# Autodesk Inventor assembly: FrameV2
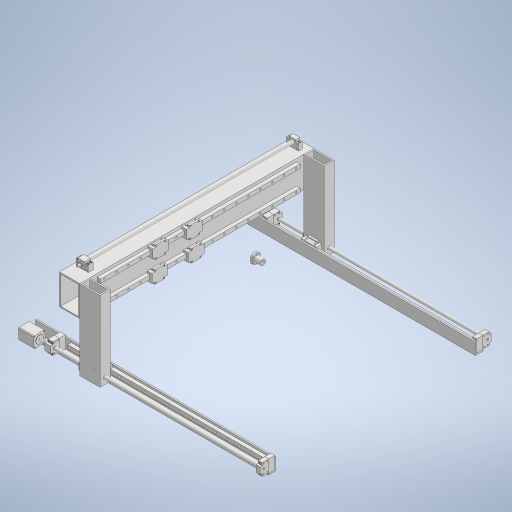
[picture p0: Inventor's stored thumbnail of the model, 512x512]
Saved by Autodesk Inventor 2023 (Build 270158000, 158)
## iProperties
Created: 2022-05-01
Part Number: FrameV2
Document SubType Name: Assembly
Designer: plebbb
Author: plebbb
## Documents named in this file (14)
- D:\Users\plebbb\Desktop\CNC_Project\FrameV2.iam
- D:\Users\plebbb\Desktop\CNC_Project\HGW20CC_Rail_800mm.ipt
- D:\Users\plebbb\Desktop\CNC_Project\HGW20CC_Slider.ipt
- D:\Users\plebbb\Desktop\CNC_Project\SFU1605_800mm.ipt
- D:\Users\plebbb\Desktop\CNC_Project\SFU1605_Nut.ipt
- D:\Users\plebbb\Desktop\CNC_Project\BF12.ipt
- D:\Users\plebbb\Desktop\CNC_Project\BK12.ipt
- D:\Users\plebbb\Desktop\CNC_Project\VERTICALTUBE.ipt
- D:\Users\plebbb\Desktop\CNC_Project\Steel_L_Bracket.ipt
- D:\Users\plebbb\Desktop\CNC_Project\BF12_Spacer.ipt
- D:\Users\plebbb\Desktop\CNC_Project\BK12_Spacer.ipt
- D:\Users\plebbb\Desktop\CNC_Project\Nema23.ipt
- D:\Users\plebbb\Desktop\CNC_Project\VERTICALTUBE_Reverse.ipt
- D:\Users\plebbb\Desktop\CNC_Project\HORIZONTALTUBE.ipt
## Components (33 placed, 13 different names)
1. VERTICALTUBE_Reverse:1 — Mate:64, Mate:65, Mate:66, Mate:72, Mate:76, Mate:79, Mate:83
2. Steel_L_Bracket:2 — Flush:25, Mate:48, Mate:52, Flush:52, Angle:3, Flush:54, Flush:55, Mate:67, Flush:56, Flush:57, Mate:77
3. HGW20CC_Rail_800mm:2 — Flush:25, Mate:48, Mate:59, Mate:60, Mate:75
4. BK12_Spacer:2 — Mate:52, Flush:52, Mate:56, Mate:57, Mate:58
5. BF12:2 — Mate:62, Mate:68, Mate:69, Mate:70, Mate:72
6. BK12:2 — Mate:56, Mate:57, Mate:58, Mate:61, Flush:53
7. SFU1605_800mm:2 — Mate:61, Flush:53, Mate:62, Mate:63, Mate:64, Mate:71, Mate:73, Mate:74
8. HGW20CC_Slider:3 — Mate:59, Mate:60, Mate:76
9. SFU1605_Nut:2 — Mate:63, Angle:3, Mate:65, Mate:66, Mate:71
10. BF12_Spacer:2 — Flush:54, Flush:55, Mate:67, Mate:68, Mate:69, Mate:70, Mate:75
11. Nema23:2 — Mate:73, Mate:74
12. HGW20CC_Rail_800mm:3 — Mate:80, Mate:82, Angle:4, Angle:5, Mate:83, Flush:60, Mate:88, Mate:89, Mate:90, Mate:91, Flush:65, Flush:66
13. HGW20CC_Rail_800mm:4 — Mate:81, Mate:82, Angle:4, Flush:60, Flush:61, Mate:84, Mate:85, Mate:86, Mate:87, Flush:62, Flush:64
14. HORIZONTALTUBE:1 — Mate:78, Mate:79, Flush:58, Flush:59, Mate:80, Mate:81, Angle:5, Flush:61, Mate:94, Flush:68, Flush:69, Mate:95
15. HGW20CC_Slider:4 — Mate:84, Mate:85, Flush:62, Mate:92
16. HGW20CC_Slider:5 — Mate:86, Mate:87, Mate:92, Flush:64
17. HGW20CC_Slider:6 — Mate:88, Mate:90, Mate:93, Flush:66
18. HGW20CC_Slider:7 — Mate:89, Mate:91, Flush:65, Mate:93
19. BF12:3 — Flush:67, Mate:94, Flush:68, Mate:96, Mate:97
20. BK12:3 — Flush:69, Mate:95, Mate:98
21. SFU1605_800mm:3 — Mate:96, Mate:97, Mate:98
22. SFU1605_Nut:3
23. HGW20CC_Rail_800mm:1 — Mate:3, Mate:4, Flush:1, Flush:21, Mate:35, Mate:38
24. SFU1605_800mm:1 — Mate:9, Mate:16, Flush:19, Mate:17, Mate:18, Mate:32, Mate:44, Mate:46, Mate:47
25. SFU1605_Nut:1 — Mate:9, Mate:33, Mate:34, Mate:44
26. HGW20CC_Slider:2 — Mate:3, Mate:4, Flush:1, Mate:25, Mate:30, Mate:31
27. BF12:1 — Mate:17, Mate:18, Angle:1, Mate:37, Mate:45
28. BK12:1 — Mate:16, Flush:19, Angle:2, Mate:40, Mate:41
29. VERTICALTUBE:1 — Mate:25, Mate:30, Mate:31, Mate:32, Mate:33, Mate:34, Mate:45, Mate:78, Flush:58, Flush:59, Flush:67
30. Steel_L_Bracket:1 — Flush:21, Mate:35, Angle:1, Mate:36, Flush:22, Flush:23, Angle:2, Mate:39, Flush:24, Flush:63, Mate:43, Flush:56, Flush:57, Mate:77
31. BF12_Spacer:1 — Mate:36, Flush:22, Flush:23, Mate:37, Mate:38
32. BK12_Spacer:1 — Mate:39, Flush:24, Mate:40, Mate:41
33. Nema23:1 — Mate:46, Mate:47
## Relationships (99: Mate 69, Flush 25, Angle 5)
- Mate:3: HGW20CC_Rail_800mm:1 ↔ HGW20CC_Slider:2
- Mate:4: HGW20CC_Rail_800mm:1 ↔ HGW20CC_Slider:2
- Mate:9: SFU1605_800mm:1 ↔ SFU1605_Nut:1
- Flush:1: HGW20CC_Rail_800mm:1 ↔ HGW20CC_Slider:2
- Mate:16: SFU1605_800mm:1 ↔ BK12:1
- Flush:19: SFU1605_800mm:1 ↔ BK12:1
- Mate:17: SFU1605_800mm:1 ↔ BF12:1
- Mate:18: SFU1605_800mm:1 ↔ BF12:1
- Mate:25: HGW20CC_Slider:2 ↔ VERTICALTUBE:1
- Mate:30: HGW20CC_Slider:2 ↔ VERTICALTUBE:1
- Mate:31: HGW20CC_Slider:2 ↔ VERTICALTUBE:1
- Mate:32: SFU1605_800mm:1 ↔ VERTICALTUBE:1
- Mate:33: SFU1605_Nut:1 ↔ VERTICALTUBE:1
- Mate:34: SFU1605_Nut:1 ↔ VERTICALTUBE:1
- Flush:21 (10 mm): HGW20CC_Rail_800mm:1 ↔ Steel_L_Bracket:1
- Mate:35: HGW20CC_Rail_800mm:1 ↔ Steel_L_Bracket:1
- Angle:1 (0 deg): BF12:1 ↔ Steel_L_Bracket:1
- Mate:36: Steel_L_Bracket:1 ↔ BF12_Spacer:1
- Flush:22: Steel_L_Bracket:1 ↔ BF12_Spacer:1
- Flush:23 (-10 mm): Steel_L_Bracket:1 ↔ BF12_Spacer:1
- Mate:37: BF12:1 ↔ BF12_Spacer:1
- Angle:2 (0 deg): BK12:1 ↔ Steel_L_Bracket:1
- Mate:38: HGW20CC_Rail_800mm:1 ↔ BF12_Spacer:1
- Mate:39: Steel_L_Bracket:1 ↔ BK12_Spacer:1
- Flush:24 (-10 mm): Steel_L_Bracket:1 ↔ BK12_Spacer:1
- Mate:40: BK12:1 ↔ BK12_Spacer:1
- Mate:41: BK12:1 ↔ BK12_Spacer:1
- Flush:63: Steel_L_Bracket:1
- Mate:43: Steel_L_Bracket:1
- Mate:44: SFU1605_800mm:1 ↔ SFU1605_Nut:1
- Mate:45: BF12:1 ↔ VERTICALTUBE:1
- Mate:46: SFU1605_800mm:1 ↔ Nema23:1
- Mate:47: SFU1605_800mm:1 ↔ Nema23:1
- Flush:25 (10 mm): Steel_L_Bracket:2 ↔ HGW20CC_Rail_800mm:2
- Mate:48: Steel_L_Bracket:2 ↔ HGW20CC_Rail_800mm:2
- Mate:52: Steel_L_Bracket:2 ↔ BK12_Spacer:2
- Flush:52 (10 mm): Steel_L_Bracket:2 ↔ BK12_Spacer:2
- Mate:56: BK12_Spacer:2 ↔ BK12:2
- Mate:57: BK12_Spacer:2 ↔ BK12:2
- Mate:58: BK12_Spacer:2 ↔ BK12:2
- Mate:59: HGW20CC_Rail_800mm:2 ↔ HGW20CC_Slider:3
- Mate:60: HGW20CC_Rail_800mm:2 ↔ HGW20CC_Slider:3
- Mate:61: BK12:2 ↔ SFU1605_800mm:2
- Flush:53: BK12:2 ↔ SFU1605_800mm:2
- Mate:62: BF12:2 ↔ SFU1605_800mm:2
- Mate:63: SFU1605_800mm:2 ↔ SFU1605_Nut:2
- Mate:64: VERTICALTUBE_Reverse:1 ↔ SFU1605_800mm:2
- Angle:3 (0 deg): Steel_L_Bracket:2 ↔ SFU1605_Nut:2
- Mate:65: VERTICALTUBE_Reverse:1 ↔ SFU1605_Nut:2
- Mate:66: VERTICALTUBE_Reverse:1 ↔ SFU1605_Nut:2
- Flush:54 (-10 mm): Steel_L_Bracket:2 ↔ BF12_Spacer:2
- Flush:55: Steel_L_Bracket:2 ↔ BF12_Spacer:2
- Mate:67: Steel_L_Bracket:2 ↔ BF12_Spacer:2
- Mate:68: BF12:2 ↔ BF12_Spacer:2
- Mate:69: BF12:2 ↔ BF12_Spacer:2
- Mate:70: BF12:2 ↔ BF12_Spacer:2
- Mate:71: SFU1605_800mm:2 ↔ SFU1605_Nut:2
- Mate:72: VERTICALTUBE_Reverse:1 ↔ BF12:2
- Mate:73: SFU1605_800mm:2 ↔ Nema23:2
- Mate:74: SFU1605_800mm:2 ↔ Nema23:2
- Flush:56: Steel_L_Bracket:2 ↔ Steel_L_Bracket:1
- Mate:75: HGW20CC_Rail_800mm:2 ↔ BF12_Spacer:2
- Flush:57: Steel_L_Bracket:2 ↔ Steel_L_Bracket:1
- Mate:76: VERTICALTUBE_Reverse:1 ↔ HGW20CC_Slider:3
- Mate:77 (1000 mm): Steel_L_Bracket:2 ↔ Steel_L_Bracket:1
- Mate:78: HORIZONTALTUBE:1 ↔ VERTICALTUBE:1
- Mate:79: VERTICALTUBE_Reverse:1 ↔ HORIZONTALTUBE:1
- Flush:58: HORIZONTALTUBE:1 ↔ VERTICALTUBE:1
- Flush:59: HORIZONTALTUBE:1 ↔ VERTICALTUBE:1
- Mate:80: HGW20CC_Rail_800mm:3 ↔ HORIZONTALTUBE:1
- Mate:81: HGW20CC_Rail_800mm:4 ↔ HORIZONTALTUBE:1
- Mate:82 (85 mm): HGW20CC_Rail_800mm:3 ↔ HGW20CC_Rail_800mm:4
- Angle:4 (0 deg): HGW20CC_Rail_800mm:3 ↔ HGW20CC_Rail_800mm:4
- Angle:5 (0 deg): HGW20CC_Rail_800mm:3 ↔ HORIZONTALTUBE:1
- Mate:83 (36.35 mm): VERTICALTUBE_Reverse:1 ↔ HGW20CC_Rail_800mm:3
- Flush:60: HGW20CC_Rail_800mm:3 ↔ HGW20CC_Rail_800mm:4
- Flush:61 (15 mm): HGW20CC_Rail_800mm:4 ↔ HORIZONTALTUBE:1
- Mate:84: HGW20CC_Rail_800mm:4 ↔ HGW20CC_Slider:4
- Mate:85: HGW20CC_Rail_800mm:4 ↔ HGW20CC_Slider:4
- Mate:86: HGW20CC_Rail_800mm:4 ↔ HGW20CC_Slider:5
- Mate:87: HGW20CC_Rail_800mm:4 ↔ HGW20CC_Slider:5
- Mate:88: HGW20CC_Rail_800mm:3 ↔ HGW20CC_Slider:6
- Mate:89: HGW20CC_Rail_800mm:3 ↔ HGW20CC_Slider:7
- Mate:90: HGW20CC_Rail_800mm:3 ↔ HGW20CC_Slider:6
- Mate:91: HGW20CC_Rail_800mm:3 ↔ HGW20CC_Slider:7
- Flush:62: HGW20CC_Rail_800mm:4 ↔ HGW20CC_Slider:4
- Mate:92: HGW20CC_Slider:4 ↔ HGW20CC_Slider:5
- Flush:64: HGW20CC_Rail_800mm:4 ↔ HGW20CC_Slider:5
- Flush:65: HGW20CC_Rail_800mm:3 ↔ HGW20CC_Slider:7
- Mate:93: HGW20CC_Slider:6 ↔ HGW20CC_Slider:7
- Flush:66: HGW20CC_Rail_800mm:3 ↔ HGW20CC_Slider:6
- Flush:67: BF12:3 ↔ VERTICALTUBE:1
- Mate:94: HORIZONTALTUBE:1 ↔ BF12:3
- Flush:68 (-15 mm): HORIZONTALTUBE:1 ↔ BF12:3
- Flush:69 (15 mm): HORIZONTALTUBE:1 ↔ BK12:3
- Mate:95: HORIZONTALTUBE:1 ↔ BK12:3
- Mate:96: BF12:3 ↔ SFU1605_800mm:3
- Mate:97: BF12:3 ↔ SFU1605_800mm:3
- Mate:98: BK12:3 ↔ SFU1605_800mm:3
